# Autodesk Inventor assembly: Mains Inlet Foot
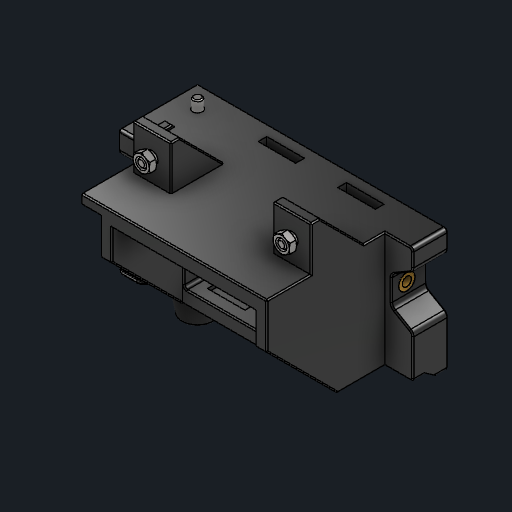
[picture p0: Inventor's stored thumbnail of the model, 512x512]
Saved by Autodesk Inventor 2026.1 (Build 301233020, 233B)
## iProperties
Created: 2025-05-09
Part Number: Mains Inlet Foot
Document SubType Name: Assembly
Designer: AdminForWorker
Title: Mains Inlet Foot
Author: AdminForWorker
## Documents named in this file (11)
- C:\Users\JoshuaEah\Documents\GitHub\Voron-0\CAD\Skirt\Feet\Mains Inlet Foot.iam
- C:\Users\JoshuaEah\Documents\GitHub\Voron-0\CAD\Skirt\Feet\Mains Inlet.ipt
- C:\Users\JoshuaEah\Documents\GitHub\Voron-0\CAD\Skirt\Feet\Rubber Foot.ipt
- C:\Users\JoshuaEah\Documents\GitHub\Voron-0\CAD\Hardware\M2x10 Self Tapper.ipt
- C:\Users\JoshuaEah\Documents\GitHub\Voron-0\CAD\Hardware\M3x10 BHCS.ipt
- C:\Users\JoshuaEah\Documents\GitHub\Voron-0\CAD\Hardware\M3x40 BHCS.ipt
- C:\Users\JoshuaEah\Documents\GitHub\Voron-0\CAD\Hardware\M3 Hexnut.ipt
- C:\Users\JoshuaEah\Documents\GitHub\Voron-0\CAD\Hardware\M3 Threaded Insert.ipt
- C:\Users\JoshuaEah\Documents\GitHub\Voron-0\CAD\Skirt\Feet\Mains Inlet Foot (1) (1).ipt
- C:\Users\JoshuaEah\Documents\GitHub\Voron-0\CAD\Skirt\Feet\Foot Accent Mirrored.ipt
- Foot Accent Left.ipt
## Components (14 placed, 9 different names)
1. Mains Inlet:1
2. Rubber Foot:2
3. M2x10 Self Tapper:1
4. M2x10 Self Tapper:2
5. M3x10 BHCS:1
6. M3x10 BHCS:2
7. M3x10 BHCS:3
8. M3x40 BHCS:1
9. M3 Hexnut:1
10. M3 Hexnut:2
11. M3 Threaded Insert:1
12. M3 Threaded Insert:2
13. Foot Accent:1
14. Mains Inlet Foot (1) (1):1
## Relationships (2: Insert 2)
- [Insert]: M2x10 Self Tapper:1 ↔ Foot Accent:1
- [Insert]: M2x10 Self Tapper:2 ↔ Foot Accent:1
